# Autodesk Inventor assembly: Wheel on a Stick
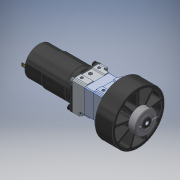
[picture p0: Inventor's stored thumbnail of the model, 180x180]
Saved by Autodesk Inventor 2018 (Build 220112000, 112)
## iProperties
Created: 2020-01-28
Part Number: Wheel on a Stick
Document SubType Name: Assembly
Designer: maste
Author: maste
## Documents named in this file (5)
- C:\Users\maste\OneDrive\Documents\GitHub\2020CAD\Control panel spinny boi\Main Assembly File\Wheel on a Stick.iam
- C:\Users\maste\OneDrive\Documents\GitHub\2020CAD\Control panel spinny boi\Part Files\VersaPlanetary_v2_Single_Stage_10_1_with_775_Series.iam
- C:\Users\maste\OneDrive\Documents\GitHub\2020CAD\Control panel spinny boi\Part Files\am-3945 3IN 500Hex Compliant Wheel VER 3.ipt
- C:\Users\maste\OneDrive\Documents\GitHub\2020CAD\Control panel spinny boi\Part Files\am-1526 500Hex HD Collar Clamp.iam
- C:\Users\maste\OneDrive\Documents\GitHub\2020CAD\Control panel spinny boi\Part Files\0.0625 Hex Spacer.ipt
## Components (4 placed, 4 different names)
1. VersaPlanetary_v2_Single_Stage_10_1_with_775_Series:1 [sub-assembly] — Mate:1, Mate:2, Mate:3, Mate:4, Flush:1, Mate:6, Mate:7, Mate:8
2. am-3945 3IN 500Hex Compliant Wheel VER 3:1 — Mate:1, Mate:2, Mate:5
3. am-1526 500Hex HD Collar Clamp:1 [sub-assembly] — Mate:3, Mate:4, Flush:1, Mate:5
4. 0.0625 Hex Spacer:1 — Mate:6, Mate:7, Mate:8
## Relationships (9: Mate 8, Flush 1)
- Mate:1: VersaPlanetary_v2_Single_Stage_10_1_with_775_Series:1 ↔ am-3945 3IN 500Hex Compliant Wheel VER 3:1
- Mate:2: VersaPlanetary_v2_Single_Stage_10_1_with_775_Series:1 ↔ am-3945 3IN 500Hex Compliant Wheel VER 3:1
- Mate:3: VersaPlanetary_v2_Single_Stage_10_1_with_775_Series:1 ↔ am-1526 500Hex HD Collar Clamp:1
- Mate:4: VersaPlanetary_v2_Single_Stage_10_1_with_775_Series:1 ↔ am-1526 500Hex HD Collar Clamp:1
- Flush:1: VersaPlanetary_v2_Single_Stage_10_1_with_775_Series:1 ↔ am-1526 500Hex HD Collar Clamp:1
- Mate:5: am-3945 3IN 500Hex Compliant Wheel VER 3:1 ↔ am-1526 500Hex HD Collar Clamp:1
- Mate:6: VersaPlanetary_v2_Single_Stage_10_1_with_775_Series:1 ↔ 0.0625 Hex Spacer:1
- Mate:7: VersaPlanetary_v2_Single_Stage_10_1_with_775_Series:1 ↔ 0.0625 Hex Spacer:1
- Mate:8: VersaPlanetary_v2_Single_Stage_10_1_with_775_Series:1 ↔ 0.0625 Hex Spacer:1
